# Autodesk Inventor assembly: Rahmen_Dreieck
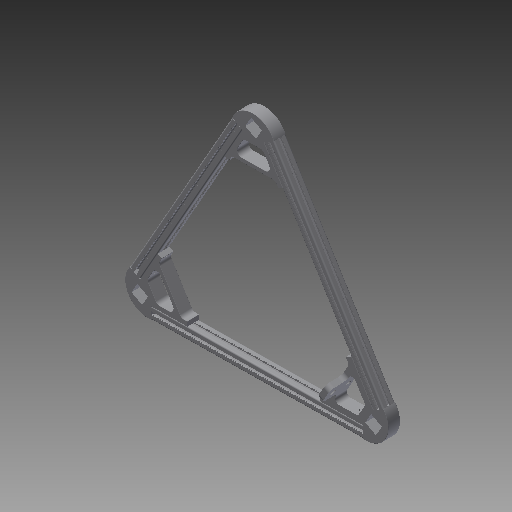
[picture p0: Inventor's stored thumbnail of the model, 512x512]
Saved by Autodesk Inventor 2019 (Build 230136000, 136)
## iProperties
Created: 2018-08-19
Part Number: Rahmen_Dreieck
Document SubType Name: Assembly
Designer: Julia
Author: Julia
## Documents named in this file (4)
- C:\Users\Julia\Documents\Inventor\3d_Drucker_v04_Single_Y_Fuehrung\Rahmen_Dreieck.iam
- C:\Users\Julia\Documents\Inventor\3d_Drucker_v04_Single_Y_Fuehrung\Rahmen_Winkel.ipt
- C:\Users\Julia\Documents\Inventor\3d_Drucker_v04_Single_Y_Fuehrung\Rahmen_Alu_Profil_Dreieck.ipt
- C:\Users\Julia\Documents\Inventor\3d_Drucker_v04_Single_Y_Fuehrung\Rahmen_Winkel_oben.ipt
## Components (6 placed, 3 different names)
1. Rahmen_Winkel:1 — Mate:1, Mate:2, Mate:3, Mate:4, Mate:5, Mate:6
2. Rahmen_Alu_Profil_Dreieck:1 — Mate:1, Mate:2, Mate:4, Mate:13
3. Rahmen_Alu_Profil_Dreieck:2 — Mate:3, Mate:5, Mate:6, Mate:7, Mate:8, Mate:9
4. Rahmen_Winkel:2 — Mate:7, Mate:8, Mate:9, Mate:10, Mate:11, Mate:12
5. Rahmen_Alu_Profil_Dreieck:3 — Mate:10, Mate:11, Mate:12, Mate:14
6. Rahmen_Winkel_oben:1 — Mate:13, Mate:14
## Relationships (14: Mate 14)
- Mate:1: Rahmen_Winkel:1 ↔ Rahmen_Alu_Profil_Dreieck:1
- Mate:2: Rahmen_Winkel:1 ↔ Rahmen_Alu_Profil_Dreieck:1
- Mate:3: Rahmen_Winkel:1 ↔ Rahmen_Alu_Profil_Dreieck:2
- Mate:4: Rahmen_Winkel:1 ↔ Rahmen_Alu_Profil_Dreieck:1
- Mate:5: Rahmen_Winkel:1 ↔ Rahmen_Alu_Profil_Dreieck:2
- Mate:6: Rahmen_Winkel:1 ↔ Rahmen_Alu_Profil_Dreieck:2
- Mate:7: Rahmen_Alu_Profil_Dreieck:2 ↔ Rahmen_Winkel:2
- Mate:8: Rahmen_Alu_Profil_Dreieck:2 ↔ Rahmen_Winkel:2
- Mate:9: Rahmen_Alu_Profil_Dreieck:2 ↔ Rahmen_Winkel:2
- Mate:10: Rahmen_Winkel:2 ↔ Rahmen_Alu_Profil_Dreieck:3
- Mate:11: Rahmen_Winkel:2 ↔ Rahmen_Alu_Profil_Dreieck:3
- Mate:12: Rahmen_Winkel:2 ↔ Rahmen_Alu_Profil_Dreieck:3
- Mate:13: Rahmen_Alu_Profil_Dreieck:1 ↔ Rahmen_Winkel_oben:1
- Mate:14: Rahmen_Alu_Profil_Dreieck:3 ↔ Rahmen_Winkel_oben:1
